# Autodesk Inventor assembly: totaal auto
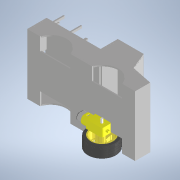
[picture p0: Inventor's stored thumbnail of the model, 180x180]
Saved by Autodesk Inventor 2021 (Build 250183000, 183)
## iProperties
Created: 2022-02-01
Part Number: totaal auto
Document SubType Name: Assembly
Designer: ryan
Author: ryan
## Documents named in this file (13)
- C:\Users\ryan\Desktop\git\projecten\school-P2-auto\modellen\inventor\auto moddellen nieuwste\totaal auto.iam
- C:\Users\ryan\Desktop\git\projecten\school-P2-auto\modellen\inventor\auto moddellen nieuwste\onderkant.ipt
- C:\Users\ryan\Desktop\git\projecten\school-P2-auto\modellen\inventor\auto moddellen nieuwste\zijplaat.ipt
- C:\Users\ryan\Desktop\git\projecten\school-P2-auto\modellen\inventor\geared-dc-motor-for-arduino-applications-1.snapshot.2\Hobi - Motor DC 1.ipt
- C:\Users\ryan\Desktop\git\projecten\school-P2-auto\modellen\inventor\wheel-arduino-1.snapshot.2\Wheel ALL.ipt
- C:\Users\ryan\Desktop\git\projecten\school-P2-auto\modellen\inventor\auto moddellen nieuwste\voorkant.ipt
- C:\Users\ryan\Desktop\git\projecten\school-P2-auto\modellen\inventor\auto moddellen nieuwste\motorkap.ipt
- C:\Users\ryan\Desktop\git\projecten\school-P2-auto\modellen\inventor\auto moddellen nieuwste\voorruit.ipt
- C:\Users\ryan\Desktop\git\projecten\school-P2-auto\modellen\inventor\auto moddellen nieuwste\dak.ipt
- C:\Users\ryan\Desktop\git\projecten\school-P2-auto\modellen\inventor\auto moddellen nieuwste\ACHTERRUIT.ipt
- C:\Users\ryan\Desktop\git\projecten\school-P2-auto\modellen\inventor\auto moddellen nieuwste\ACHTERKANT.ipt
- C:\Users\ryan\Desktop\git\projecten\school-P2-auto\modellen\inventor\auto moddellen nieuwste\achterbak.ipt
- C:\Users\ryan\Desktop\git\projecten\school-P2-auto\modellen\inventor\auto moddellen nieuwste\krat houder.iam
## Components (14 placed, 12 different names)
1. onderkant:1 — Flush:1, Mate:1, Flush:2, Flush:3, Mate:3, Flush:4, Flush:5, Flush:6, Flush:7, Mate:4
2. zijplaat:1 — Flush:1, Mate:3, Flush:4, Flush:5, Flush:8, Flush:14, Flush:15, Flush:17, Flush:18, Flush:20, Flush:21, Flush:22, Flush:23, Flush:28
3. Hobi - Motor DC 1:1 — Mate:1, Flush:2, Mate:2
4. Wheel ALL:1 — Mate:2
5. voorkant:1 — Flush:3, Flush:6, Flush:7, Flush:8, Flush:9, Flush:10
6. zijplaat:2 — Flush:9, Flush:10, Mate:4, Flush:11, Flush:12, Flush:13, Flush:16, Flush:24, Flush:26
7. motorkap:1 — Flush:11, Flush:12, Flush:13
8. voorruit:1 — Flush:14, Flush:21, Flush:22
9. dak:1 — Flush:15, Flush:19, Flush:20
10. ACHTERRUIT:1 — Flush:16, Flush:17, Flush:18, Flush:19
11. ACHTERKANT:1 — Flush:23, Flush:25, Flush:27
12. achterbak:1 — Flush:24, Mate:5, Mate:6
13. krat houder:1 [sub-assembly] — Flush:27, Flush:28, Mate:6
14. krat houder:2 [sub-assembly] — Mate:5, Flush:25, Flush:26
## Relationships (34: Flush 28, Mate 6)
- Flush:1: onderkant:1 ↔ zijplaat:1
- Mate:1: onderkant:1 ↔ Hobi - Motor DC 1:1
- Flush:2: onderkant:1 ↔ Hobi - Motor DC 1:1
- Mate:2: Hobi - Motor DC 1:1 ↔ Wheel ALL:1
- Flush:3: onderkant:1 ↔ voorkant:1
- Mate:3: onderkant:1 ↔ zijplaat:1
- Flush:4: onderkant:1 ↔ zijplaat:1
- Flush:5: onderkant:1 ↔ zijplaat:1
- Flush:6: onderkant:1 ↔ voorkant:1
- Flush:7: onderkant:1 ↔ voorkant:1
- Flush:8: zijplaat:1 ↔ voorkant:1
- Flush:9: voorkant:1 ↔ zijplaat:2
- Flush:10: voorkant:1 ↔ zijplaat:2
- Mate:4: onderkant:1 ↔ zijplaat:2
- Flush:11: zijplaat:2 ↔ motorkap:1
- Flush:12: zijplaat:2 ↔ motorkap:1
- Flush:13: zijplaat:2 ↔ motorkap:1
- Flush:14: zijplaat:1 ↔ voorruit:1
- Flush:15: zijplaat:1 ↔ dak:1
- Flush:16: zijplaat:2 ↔ ACHTERRUIT:1
- Flush:17: zijplaat:1 ↔ ACHTERRUIT:1
- Flush:18: zijplaat:1 ↔ ACHTERRUIT:1
- Flush:19: dak:1 ↔ ACHTERRUIT:1
- Flush:20: zijplaat:1 ↔ dak:1
- Flush:21: zijplaat:1 ↔ voorruit:1
- Flush:22: zijplaat:1 ↔ voorruit:1
- Flush:23: zijplaat:1 ↔ ACHTERKANT:1
- Flush:24: zijplaat:2 ↔ achterbak:1
- Mate:5: achterbak:1 ↔ krat houder:2
- Flush:25: ACHTERKANT:1 ↔ krat houder:2
- Flush:26: zijplaat:2 ↔ krat houder:2
- Flush:27: ACHTERKANT:1 ↔ krat houder:1
- Flush:28: zijplaat:1 ↔ krat houder:1
- Mate:6: achterbak:1 ↔ krat houder:1
